# Autodesk Inventor assembly: arm
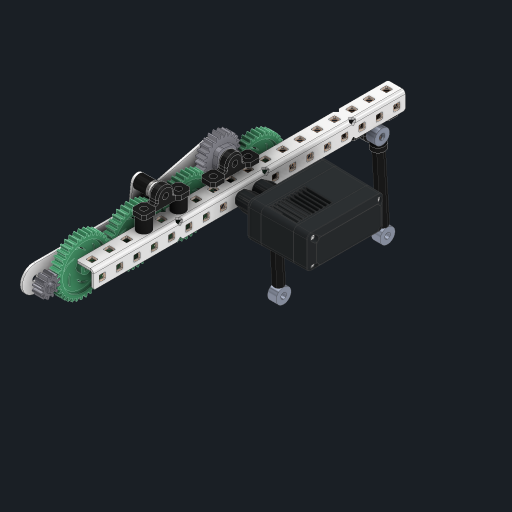
[picture p0: Inventor's stored thumbnail of the model, 512x512]
Saved by Autodesk Inventor 2024 (Build 280153000, 153)
## iProperties
Created: 2023-08-20
Part Number: arm
Document SubType Name: Assembly
Designer: Averey
Author: Averey
## Documents named in this file (21)
- D:\vex_robotics\hardware\cad\scrap_v0.1\intake\arm.iam
- D:\vex_robotics\hardware\cad\VEX-CAD-Inventor-1.41\Structure\Angle\Aluminum 1x1\Alu Angle 1x1x18.ipt
- D:\vex_robotics\hardware\cad\VEX-CAD-Inventor-1.41\Motion\Spacers\Spacer Nylon .375 OD\NSpacer .375 OD x .375.ipt
- D:\vex_robotics\hardware\cad\VEX-CAD-Inventor-1.41\Motion\Shaft LS\LS Pillow Bearing Block.ipt
- D:\vex_robotics\hardware\cad\VEX-CAD-Inventor-1.41\Motion\Shaft LS\Shaft Collar ipts\Shaft Collar No Screw.ipt
- D:\vex_robotics\hardware\cad\VEX-CAD-Inventor-1.41\Motion\Spacers\Washer Steel\SWasher .375 OD x .062500.ipt
- D:\vex_robotics\hardware\cad\VEX-CAD-Inventor-1.41\Motion\Gears\LS 36T Gear.ipt
- D:\vex_robotics\hardware\cad\scrap_v0.1\catapult\custom_parts\half_cut_24.ipt
- D:\vex_robotics\hardware\cad\scrap_v0.1\intake\custom_parts\intake_gusset.ipt
- D:\vex_robotics\hardware\cad\VEX-CAD-Inventor-1.41\Structure\Standoff\Standoff .875.ipt
- D:\vex_robotics\hardware\cad\VEX-CAD-Inventor-1.41\Motion\Spacers\Washer Steel\SWasher .375 OD x .015625.ipt
- D:\vex_robotics\hardware\cad\VEX-CAD-Inventor-1.41\Motion\Spacers\Washer Steel\SWasher .375 OD x .031250.ipt
- D:\vex_robotics\hardware\cad\VEX-CAD-Inventor-1.41\Motion\Spacers\Washer Teflon\TWasher .375 OD x .04000.ipt
- D:\vex_robotics\hardware\cad\VEX-CAD-Inventor-1.41\Motion\Gears\LS 12T Gear Steel.ipt
- D:\vex_robotics\hardware\cad\VEX-CAD-Inventor-1.41\Electronics\V5 Motor (5.5W).ipt
- D:\vex_robotics\hardware\cad\VEX-CAD-Inventor-1.41\Motion\Spacers\Spacer Nylon .375 OD.ipt
- D:\vex_robotics\hardware\cad\VEX-CAD-Inventor-1.41\Motion\Spacers\Washer Steel.ipt
- D:\vex_robotics\hardware\cad\VEX-CAD-Inventor-1.41\Structure\Standoff.ipt
- D:\vex_robotics\hardware\cad\VEX-CAD-Inventor-1.41\Motion\Spacers\Washer Teflon.ipt
- D:\vex_robotics\hardware\cad\VEX-CAD-Inventor-1.41\Motion\Spacers\Spacer Nylon .375 OD\NSpacer .375 OD x .125.ipt
- D:\vex_robotics\hardware\cad\VEX-CAD-Inventor-1.41\Structure\Standoff\Standoff 2.00.ipt
## Components (38 placed, 16 different names)
1. Alu Angle 1x1x18:2 — Insert:1, Insert:2, Insert:15, Insert:16, Insert:26, Insert:29, Insert:34, Insert:35, Mate:4, Insert:44, Mate:8, Insert:64, Insert:65, Insert:70, Mate:13, Insert:71
2. NSpacer .375 OD x .375:1 — Insert:1, Insert:3
3. NSpacer .375 OD x .375:2 — Insert:2, Insert:4
4. LS Pillow Bearing Block:1 — Insert:5, Mate:1, Insert:6
5. Shaft Collar No Screw:1 — Insert:6, Flush:1, Insert:77
6. Shaft Collar No Screw:2 — Flush:1, Insert:78
7. SWasher .375 OD x .062500:1 — Insert:3, Insert:5
8. SWasher .375 OD x .062500:2 — Insert:4, Mate:1
9. NSpacer .375 OD x .375:3 — Insert:15
10. NSpacer .375 OD x .375:4 — Insert:16
11. LS Pillow Bearing Block:2
12. Shaft Collar No Screw:3 — Insert:74
13. Shaft Collar No Screw:4 — Insert:75
14. SWasher .375 OD x .062500:3
15. SWasher .375 OD x .062500:4
16. LS 36T Gear:1 — Insert:26
17. LS 36T Gear:2 — Insert:29
18. LS 36T Gear:3 — Insert:34, Insert:43
19. LS Pillow Bearing Block:3 — Insert:35, Mate:4, Insert:36
20. half_cut_24:1 — Insert:36
21. intake_gusset:1 — Insert:43, Insert:63, Insert:72, Mate:14
22. Standoff .875:5 — Insert:44
23. LS Pillow Bearing Block:4 — Mate:8, Mate:9, Insert:66, Mate:11
24. SWasher .375 OD x .015625:6 — Insert:66, Insert:67
25. SWasher .375 OD x .015625:8 — Mate:9, Insert:68, Mate:11
26. NSpacer .375 OD x .375:7 — Insert:53, Insert:63
27. SWasher .375 OD x .062500:9 — Insert:51, Insert:53
28. SWasher .375 OD x .031250:10 — Insert:52
29. TWasher .375 OD x .04000:1 — Insert:51, Insert:52
30. NSpacer .375 OD x .375:8 — Insert:64, Insert:67
31. NSpacer .375 OD x .375:9 — Insert:65, Insert:68
32. V5 Motor (5.5W):1 — Insert:70, Mate:13
33. LS 36T Gear:4 — Insert:71, Mate:14
34. LS 12T Gear Steel:1 — Insert:72
35. NSpacer .375 OD x .125:10 — Insert:73, Insert:74
36. Standoff 2.00:8 — Insert:73, Insert:75
37. NSpacer .375 OD x .125:11 — Insert:77
38. Standoff 2.00:9 — Insert:78
## Relationships (47: Insert 37, Mate 8, Flush 2)
- Insert:1: Alu Angle 1x1x18:2 ↔ NSpacer .375 OD x .375:1
- Insert:2: Alu Angle 1x1x18:2 ↔ NSpacer .375 OD x .375:2
- Insert:3: NSpacer .375 OD x .375:1 ↔ SWasher .375 OD x .062500:1
- Insert:4: NSpacer .375 OD x .375:2 ↔ SWasher .375 OD x .062500:2
- Insert:5: LS Pillow Bearing Block:1 ↔ SWasher .375 OD x .062500:1
- Mate:1: LS Pillow Bearing Block:1 ↔ SWasher .375 OD x .062500:2
- Insert:6: LS Pillow Bearing Block:1 ↔ Shaft Collar No Screw:1
- Flush:1: Shaft Collar No Screw:1 ↔ Shaft Collar No Screw:2
- [Insert]: NSpacer .375 OD x .375:3 ↔ SWasher .375 OD x .062500:3
- [Insert]: NSpacer .375 OD x .375:4 ↔ SWasher .375 OD x .062500:4
- [Insert]: LS Pillow Bearing Block:2 ↔ SWasher .375 OD x .062500:3
- [Mate]: LS Pillow Bearing Block:2 ↔ SWasher .375 OD x .062500:4
- [Insert]: LS Pillow Bearing Block:2 ↔ Shaft Collar No Screw:3
- [Flush]: Shaft Collar No Screw:3 ↔ Shaft Collar No Screw:4
- Insert:15: Alu Angle 1x1x18:2 ↔ NSpacer .375 OD x .375:3
- Insert:16: Alu Angle 1x1x18:2 ↔ NSpacer .375 OD x .375:4
- Insert:26 (9.9219 mm): Alu Angle 1x1x18:2 ↔ LS 36T Gear:1
- Insert:29 (9.9219 mm): Alu Angle 1x1x18:2 ↔ LS 36T Gear:2
- Insert:34 (9.9219 mm): Alu Angle 1x1x18:2 ↔ LS 36T Gear:3
- Insert:35 (5.1594 mm): Alu Angle 1x1x18:2 ↔ LS Pillow Bearing Block:3
- Mate:4: Alu Angle 1x1x18:2 ↔ LS Pillow Bearing Block:3
- Insert:36: LS Pillow Bearing Block:3 ↔ half_cut_24:1
- Insert:43 (2.6035 mm): LS 36T Gear:3 ↔ intake_gusset:1
- Insert:44: Alu Angle 1x1x18:2 ↔ Standoff .875:5
- Mate:8: Alu Angle 1x1x18:2 ↔ LS Pillow Bearing Block:4
- Insert:51: SWasher .375 OD x .062500:9 ↔ TWasher .375 OD x .04000:1
- Insert:52: SWasher .375 OD x .031250:10 ↔ TWasher .375 OD x .04000:1
- Insert:53: NSpacer .375 OD x .375:7 ↔ SWasher .375 OD x .062500:9
- Mate:9: LS Pillow Bearing Block:4 ↔ SWasher .375 OD x .015625:8
- Insert:63: intake_gusset:1 ↔ NSpacer .375 OD x .375:7
- Insert:64: Alu Angle 1x1x18:2 ↔ NSpacer .375 OD x .375:8
- Insert:65: Alu Angle 1x1x18:2 ↔ NSpacer .375 OD x .375:9
- Insert:66: LS Pillow Bearing Block:4 ↔ SWasher .375 OD x .015625:6
- Insert:67: SWasher .375 OD x .015625:6 ↔ NSpacer .375 OD x .375:8
- Insert:68: SWasher .375 OD x .015625:8 ↔ NSpacer .375 OD x .375:9
- Mate:11: LS Pillow Bearing Block:4 ↔ SWasher .375 OD x .015625:8
- Insert:70: Alu Angle 1x1x18:2 ↔ V5 Motor (5.5W):1
- Mate:13: Alu Angle 1x1x18:2 ↔ V5 Motor (5.5W):1
- Insert:71 (9.9219 mm): Alu Angle 1x1x18:2 ↔ LS 36T Gear:4
- Insert:72 (3.175 mm): intake_gusset:1 ↔ LS 12T Gear Steel:1
- Mate:14: intake_gusset:1 ↔ LS 36T Gear:4
- Insert:73: NSpacer .375 OD x .125:10 ↔ Standoff 2.00:8
- Insert:74: Shaft Collar No Screw:3 ↔ NSpacer .375 OD x .125:10
- Insert:75: Shaft Collar No Screw:4 ↔ Standoff 2.00:8
- [Insert]: NSpacer .375 OD x .125:11 ↔ Standoff 2.00:9
- Insert:77: Shaft Collar No Screw:1 ↔ NSpacer .375 OD x .125:11
- Insert:78: Shaft Collar No Screw:2 ↔ Standoff 2.00:9
## Named parameters: d12_d4 = 0 mm, d13_d5 = 0 mm, d14_d6 = 0 mm, d15_d7 = 0 mm, d16_d8 = 0 mm, d19_d11 = 0 mm, d108_d105 = 0 mm
